# Autodesk Inventor assembly: END OF ARM TOOL_1
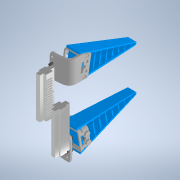
[picture p0: Inventor's stored thumbnail of the model, 180x180]
Saved by Autodesk Inventor 2020 (Build 240168000, 168)
## iProperties
Created: 2020-05-25
Part Number: END OF ARM TOOL_1
Document SubType Name: Assembly
Designer: Gebruiker
Author: Gebruiker
## Documents named in this file (3)
- C:\Users\Gebruiker\Documents\GitHub\BeerMinder\3D-model\servo\END OF ARM TOOL_1.iam
- C:\Users\Gebruiker\Documents\GitHub\BeerMinder\3D-model\servo\AGF.iam
- C:\Users\Gebruiker\Desktop\SMR\Robotarm\GripperV2_2.ipt
## Components (4 placed, 2 different names)
1. AGF:1 [sub-assembly] — Flush:1, Mate:2, Mate:3, Mate:6, Mate:7, Mate:8
2. AGF:2 [sub-assembly] — Flush:1, Mate:2, Mate:3, Mate:9, Mate:10, Mate:11
3. GripperV2_2:1 — Mate:9, Mate:10, Mate:11
4. GripperV2_2:2 — Mate:6, Mate:7, Mate:8
## Relationships (9: Mate 8, Flush 1)
- Flush:1: AGF:1 ↔ AGF:2
- Mate:2: AGF:1 ↔ AGF:2
- Mate:3 (63 mm): AGF:1 ↔ AGF:2
- Mate:6: AGF:1 ↔ GripperV2_2:2
- Mate:7: AGF:1 ↔ GripperV2_2:2
- Mate:8: AGF:1 ↔ GripperV2_2:2
- Mate:9: AGF:2 ↔ GripperV2_2:1
- Mate:10: AGF:2 ↔ GripperV2_2:1
- Mate:11: AGF:2 ↔ GripperV2_2:1
